# Autodesk Inventor assembly: Idler Pulley
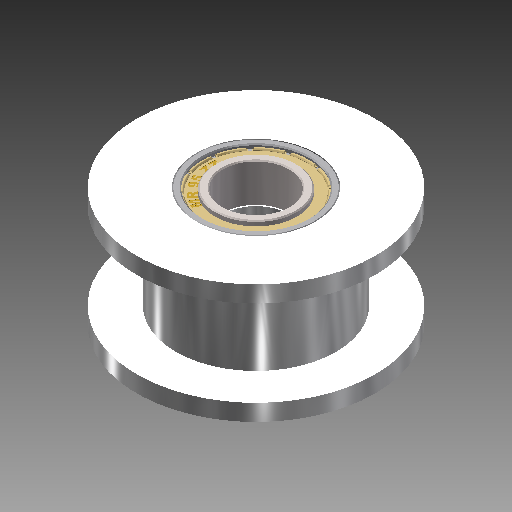
[picture p0: Inventor's stored thumbnail of the model, 512x512]
Saved by Autodesk Inventor 2019 (Build 230136000, 136)
## iProperties
Created: 2018-10-13
Part Number: Idler Pulley
Document SubType Name: Assembly
Designer: Ax
Mass: 2.68786 g
Surface Area: 22.6792 cm^2
Volume: 1.08476 cm^3
Density: 2.47784 g/cm^3
Author: Ax
## Documents named in this file (3)
- C:\Users\Ax\Google Drive\Inventor\AX-01\Idler Pulley.iam
- C:\Users\Ax\Google Drive\Inventor\AX-01\Idler Pulley.ipt
- C:\Users\Ax\Google Drive\Inventor\Library\-MR95ZZ-assem.iam
## Components (3 placed, 2 different names)
1. Idler Pulley:1 — Mate:1, Mate:2, Mate:3, Mate:4
2. -MR95ZZ-assem:1 [sub-assembly] — Mate:3, Mate:4
3. -MR95ZZ-assem:2 [sub-assembly] — Mate:1, Mate:2
## Relationships (4: Mate 4)
- Mate:1: Idler Pulley:1 ↔ -MR95ZZ-assem:2
- Mate:2: Idler Pulley:1 ↔ -MR95ZZ-assem:2
- Mate:3: Idler Pulley:1 ↔ -MR95ZZ-assem:1
- Mate:4: Idler Pulley:1 ↔ -MR95ZZ-assem:1
